# Autodesk Inventor assembly: Мостики
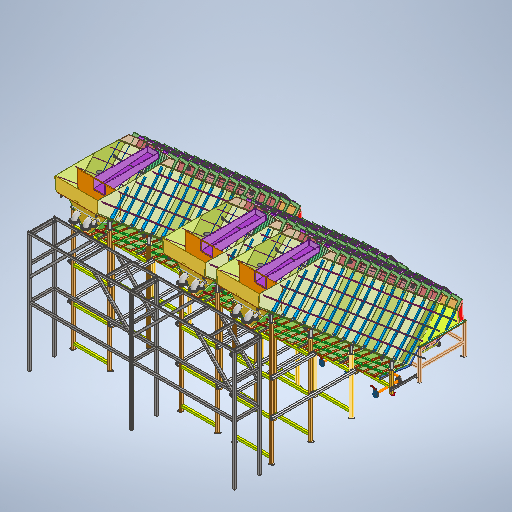
[picture p0: Inventor's stored thumbnail of the model, 512x512]
Saved by Autodesk Inventor 2025 (Build 290162010, 162A)
## iProperties
Created: 2025-01-27
Part Number: Мостики
Document SubType Name: Assembly
Designer: admin
Author: admin
## Documents named in this file (10)
- C:\Users\pokla\Documents\Inventor\Отстойник осветлитель\Manturovo_Se-clar-Gleb\Мостики.iam
- C:\Users\pokla\Documents\Inventor\Отстойник осветлитель\Manturovo_Se-clar-Gleb\ASY MSC 002 отстойник осветлитель.iam
- C:\Users\pokla\Documents\Inventor\Отстойник осветлитель\Manturovo_Se-clar-Gleb\human 01\ч ASY human dummy 01.iam
- C:\Users\pokla\Documents\Inventor\Отстойник осветлитель\Manturovo_Se-clar-Gleb\ASY MSC Платформа отстойников.iam
- C:\Users\pokla\Documents\Inventor\Отстойник осветлитель\Manturovo_Se-clar-Gleb\ASY MSC Опора №1 платф. отст..iam
- C:\Users\pokla\Documents\Inventor\Отстойник осветлитель\Manturovo_Se-clar-Gleb\ASY MSC Опора №2 платф. отст..iam
- C:\Users\pokla\Documents\Inventor\Отстойник осветлитель\Manturovo_Se-clar-Gleb\Габаритные емкости для Димы\Отстойник промывных вод.ipt
- C:\Users\pokla\Documents\Inventor\Отстойник осветлитель\Manturovo_Se-clar-Gleb\ASY MSC Усиление №1.iam
- C:\Users\pokla\Documents\Inventor\Отстойник осветлитель\Manturovo_Se-clar-Gleb\ASY MSC Усиление №2.iam
- C:\Users\pokla\Documents\Inventor\Отстойник осветлитель\Manturovo_Se-clar-Gleb\ASY MSC Мостики уголок.ipt
## Components (32 placed, 9 different names)
1. ASY MSC 002 отстойник осветлитель:1 [sub-assembly] — Flush:1, Flush:2, Flush:3, Flush:4, Rigid:1, Mate:6, Flush:22
2. ASY MSC 002 отстойник осветлитель:2 [sub-assembly] — Rigid:1, Rigid:2
3. ASY MSC 002 отстойник осветлитель:3 [sub-assembly] — Rigid:3
4. ASY MSC 002 отстойник осветлитель:4 [sub-assembly] — Rigid:2, Rigid:3
5. ч ASY human dummy 01:1 [sub-assembly] — Flush:1
6. ASY MSC Платформа отстойников:1 [sub-assembly] — Flush:6, Mate:6, Mate:15, Mate:17, Mate:20, Mate:22, Flush:21, Rigid:15, Mate:30
7. ASY MSC Опора №1 платф. отст.:1 [sub-assembly] — Flush:6, Rigid:5, Mate:5, Rigid:7, Rigid:8, Mate:16, Flush:12, Mate:19, Flush:14, Mate:25, Flush:20, Flush:21, Flush:22, Mate:30
8. ASY MSC Опора №1 платф. отст.:2 [sub-assembly] — Rigid:6, Mate:12, Flush:10, Mate:14, Flush:11
9. ASY MSC Опора №2 платф. отст.:1 [sub-assembly]
10. ASY MSC Опора №1 платф. отст.:3 [sub-assembly] — Rigid:5, Rigid:6, Rigid:9, Rigid:10, Mate:8, Flush:8, Mate:9, Flush:9, Mate:18, Flush:13, Mate:21, Flush:15, Flush:17, Flush:19
11. Отстойник промывных вод:1 — Mate:3
12. ASY MSC Платформа отстойников:2 [sub-assembly] — Rigid:15, Mate:26, Mate:27, Mate:28, Mate:29
13. ASY MSC Усиление №1:1 [sub-assembly] — Rigid:7
14. ASY MSC Усиление №1:2 [sub-assembly] — Rigid:8
15. ASY MSC Усиление №1:3 [sub-assembly] — Rigid:9
16. ASY MSC Усиление №1:4 [sub-assembly] — Rigid:10
17. ASY MSC Усиление №2:1 [sub-assembly] — Mate:8, Flush:8, Mate:26
18. ASY MSC Усиление №2:2 [sub-assembly] — Mate:9, Flush:9, Mate:27
19. ASY MSC Усиление №2:3 [sub-assembly] — Mate:12, Flush:10, Mate:28
20. ASY MSC Усиление №2:4 [sub-assembly] — Mate:14, Flush:11, Mate:29
21. ASY MSC Усиление №2:5 [sub-assembly] — Mate:15, Mate:16, Flush:12
22. ASY MSC Усиление №2:6 [sub-assembly] — Mate:17, Mate:18, Flush:13
23. ASY MSC Усиление №2:7 [sub-assembly] — Mate:19, Mate:20, Flush:14
24. ASY MSC Усиление №2:8 [sub-assembly] — Mate:21, Mate:22, Flush:15
25. ASY MSC Мостики уголок:1 — Rigid:12, Flush:17
26. ASY MSC Мостики уголок:2 — Rigid:12
27. ASY MSC Мостики уголок:3
28. ASY MSC Мостики уголок:4 — Flush:19
29. ASY MSC Мостики уголок:5 — Mate:25, Flush:20
30. ASY MSC Мостики уголок:6
31. ASY MSC Мостики уголок:7
32. ASY MSC Мостики уголок:8
## Relationships (53: Mate 21, Flush 18, WeldJoint 14)
- Flush:1 (4500 mm): ASY MSC 002 отстойник осветлитель:1 ↔ ч ASY human dummy 01:1
- Flush:2: ASY MSC 002 отстойник осветлитель:1
- Flush:3: ASY MSC 002 отстойник осветлитель:1
- Flush:4: ASY MSC 002 отстойник осветлитель:1
- Rigid:1 [WeldJoint] (300 mm): ASY MSC 002 отстойник осветлитель:1 ↔ ASY MSC 002 отстойник осветлитель:2
- Rigid:2 [WeldJoint] (300 mm): ASY MSC 002 отстойник осветлитель:2 ↔ ASY MSC 002 отстойник осветлитель:4
- Rigid:3 [WeldJoint] (300 mm): ASY MSC 002 отстойник осветлитель:3 ↔ ASY MSC 002 отстойник осветлитель:4
- Mate:3: Отстойник промывных вод:1
- Flush:6: ASY MSC Платформа отстойников:1 ↔ ASY MSC Опора №1 платф. отст.:1
- Rigid:5 [WeldJoint] (3730 mm): ASY MSC Опора №1 платф. отст.:1 ↔ ASY MSC Опора №1 платф. отст.:3
- Rigid:6 [WeldJoint] (3730 mm): ASY MSC Опора №1 платф. отст.:2 ↔ ASY MSC Опора №1 платф. отст.:3
- Mate:5: ASY MSC Опора №1 платф. отст.:1
- Mate:6 (500 mm): ASY MSC 002 отстойник осветлитель:1 ↔ ASY MSC Платформа отстойников:1
- Rigid:7 [WeldJoint]: ASY MSC Опора №1 платф. отст.:1 ↔ ASY MSC Усиление №1:1
- Rigid:8 [WeldJoint]: ASY MSC Опора №1 платф. отст.:1 ↔ ASY MSC Усиление №1:2
- Rigid:9 [WeldJoint]: ASY MSC Опора №1 платф. отст.:3 ↔ ASY MSC Усиление №1:3
- Rigid:10 [WeldJoint]: ASY MSC Опора №1 платф. отст.:3 ↔ ASY MSC Усиление №1:4
- Mate:8: ASY MSC Опора №1 платф. отст.:3 ↔ ASY MSC Усиление №2:1
- Flush:8: ASY MSC Опора №1 платф. отст.:3 ↔ ASY MSC Усиление №2:1
- Mate:9: ASY MSC Опора №1 платф. отст.:3 ↔ ASY MSC Усиление №2:2
- Flush:9: ASY MSC Опора №1 платф. отст.:3 ↔ ASY MSC Усиление №2:2
- Mate:12: ASY MSC Опора №1 платф. отст.:2 ↔ ASY MSC Усиление №2:3
- Flush:10: ASY MSC Опора №1 платф. отст.:2 ↔ ASY MSC Усиление №2:3
- Mate:14: ASY MSC Опора №1 платф. отст.:2 ↔ ASY MSC Усиление №2:4
- Flush:11: ASY MSC Опора №1 платф. отст.:2 ↔ ASY MSC Усиление №2:4
- Mate:15: ASY MSC Платформа отстойников:1 ↔ ASY MSC Усиление №2:5
- Mate:16: ASY MSC Опора №1 платф. отст.:1 ↔ ASY MSC Усиление №2:5
- Flush:12: ASY MSC Опора №1 платф. отст.:1 ↔ ASY MSC Усиление №2:5
- Mate:17: ASY MSC Платформа отстойников:1 ↔ ASY MSC Усиление №2:6
- Mate:18: ASY MSC Опора №1 платф. отст.:3 ↔ ASY MSC Усиление №2:6
- Flush:13: ASY MSC Опора №1 платф. отст.:3 ↔ ASY MSC Усиление №2:6
- Mate:19: ASY MSC Опора №1 платф. отст.:1 ↔ ASY MSC Усиление №2:7
- Mate:20: ASY MSC Платформа отстойников:1 ↔ ASY MSC Усиление №2:7
- Flush:14: ASY MSC Опора №1 платф. отст.:1 ↔ ASY MSC Усиление №2:7
- Mate:21: ASY MSC Опора №1 платф. отст.:3 ↔ ASY MSC Усиление №2:8
- Mate:22: ASY MSC Платформа отстойников:1 ↔ ASY MSC Усиление №2:8
- Flush:15: ASY MSC Опора №1 платф. отст.:3 ↔ ASY MSC Усиление №2:8
- Rigid:12 [WeldJoint]: ASY MSC Мостики уголок:1 ↔ ASY MSC Мостики уголок:2
- Flush:17: ASY MSC Опора №1 платф. отст.:3 ↔ ASY MSC Мостики уголок:1
- [WeldJoint]: ASY MSC Мостики уголок:3 ↔ ASY MSC Мостики уголок:4
- Flush:19: ASY MSC Опора №1 платф. отст.:3 ↔ ASY MSC Мостики уголок:4
- [WeldJoint]: ASY MSC Мостики уголок:5 ↔ ASY MSC Мостики уголок:6
- Mate:25: ASY MSC Опора №1 платф. отст.:1 ↔ ASY MSC Мостики уголок:5
- Flush:20: ASY MSC Опора №1 платф. отст.:1 ↔ ASY MSC Мостики уголок:5
- Flush:21: ASY MSC Платформа отстойников:1 ↔ ASY MSC Опора №1 платф. отст.:1
- Rigid:15 [WeldJoint]: ASY MSC Платформа отстойников:1 ↔ ASY MSC Платформа отстойников:2
- Mate:26: ASY MSC Платформа отстойников:2 ↔ ASY MSC Усиление №2:1
- Mate:27: ASY MSC Платформа отстойников:2 ↔ ASY MSC Усиление №2:2
- Mate:28: ASY MSC Платформа отстойников:2 ↔ ASY MSC Усиление №2:3
- Mate:29: ASY MSC Платформа отстойников:2 ↔ ASY MSC Усиление №2:4
- Flush:22: ASY MSC 002 отстойник осветлитель:1 ↔ ASY MSC Опора №1 платф. отст.:1
- Mate:30: ASY MSC Платформа отстойников:1 ↔ ASY MSC Опора №1 платф. отст.:1
- [WeldJoint]: ASY MSC Мостики уголок:7 ↔ ASY MSC Мостики уголок:8
## Named parameters: d83_d79 = 0 mm, d87_d79 = 0 mm, d98_d83_d79 = 0 mm
